# Autodesk Inventor assembly: Entire Robot
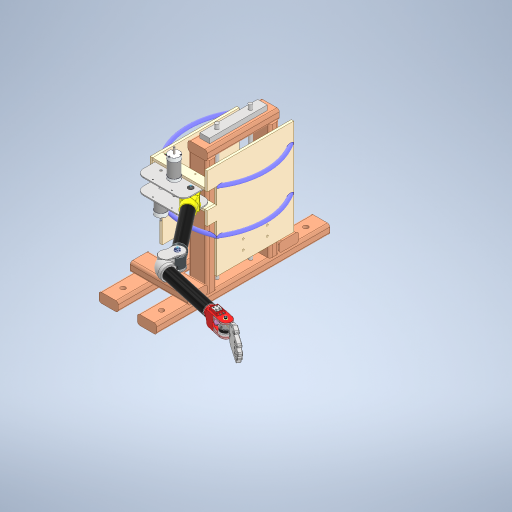
[picture p0: Inventor's stored thumbnail of the model, 512x512]
Saved by Autodesk Inventor 2024 (Build 280153000, 153)
## iProperties
Created: 2024-03-21
Part Number: Entire Robot
Document SubType Name: Assembly
Designer: Liz
Author: Liz
## Documents named in this file (4)
- C:\Users\anyangoe\Desktop\WholeRobot\Entire Robot.iam
- C:\Users\anyangoe\Desktop\WholeRobot\Height Adjustment Frame.iam
- C:\Users\anyangoe\Desktop\WholeRobot\Torso.iam
- C:\Users\anyangoe\Desktop\WholeRobot\FullAssembly.iam
## Components (3 placed, 3 different names)
1. Height Adjustment Frame:1 [sub-assembly] — Mate:1, Mate:2, Mate:3
2. Torso:1 [sub-assembly] — Mate:1, Mate:2, Mate:3, Mate:4, Mate:5, Mate:6
3. FullAssembly:1 [sub-assembly] — Mate:4, Mate:5, Mate:6
## Relationships (6: Mate 6)
- Mate:1: Height Adjustment Frame:1 ↔ Torso:1
- Mate:2: Height Adjustment Frame:1 ↔ Torso:1
- Mate:3 (50.8 mm): Height Adjustment Frame:1 ↔ Torso:1
- Mate:4: Torso:1 ↔ FullAssembly:1
- Mate:5: Torso:1 ↔ FullAssembly:1
- Mate:6: Torso:1 ↔ FullAssembly:1
